# Autodesk Inventor assembly: Vergaser_ra8846s
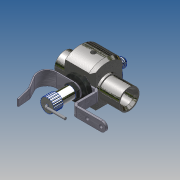
[picture p0: Inventor's stored thumbnail of the model, 180x180]
Saved by Autodesk Inventor 2021 (Build 250183000, 183)
## iProperties
Created: 2021-01-14
Part Number: Vergaser_ra8846s
Document SubType Name: Assembly
Designer: Sander
Author: Sander
## Documents named in this file (11)
- C:\Users\ricar\OneDrive - Fachhochschule Aachen\Mechatronik I\CAD\INVENTOR\Proyectos\Daten\Vergaser_ra8846s.iam
- C:\Users\ricar\OneDrive - Fachhochschule Aachen\Mechatronik I\CAD\INVENTOR\Proyectos\Daten\Vergasergehäuse_ra8846s.ipt
- C:\Users\ricar\OneDrive - Fachhochschule Aachen\Mechatronik I\CAD\INVENTOR\Proyectos\Daten\Einspritzdüse_ra8846s.ipt
- C:\Users\ricar\OneDrive - Fachhochschule Aachen\Mechatronik I\CAD\INVENTOR\Proyectos\Daten\Schließbahn_ra8846s.ipt
- C:\Users\ricar\OneDrive - Fachhochschule Aachen\Mechatronik I\CAD\INVENTOR\Proyectos\Daten\Gashebel_ra8846s.ipt
- C:\Users\ricar\OneDrive - Fachhochschule Aachen\Mechatronik I\CAD\INVENTOR\Proyectos\Daten\Dichtrign_ra8846s.ipt
- C:\Users\ricar\OneDrive - Fachhochschule Aachen\Mechatronik I\CAD\INVENTOR\Proyectos\Daten\Deckel_ra8846s.ipt
- C:\Users\ricar\OneDrive - Fachhochschule Aachen\Mechatronik I\CAD\INVENTOR\Proyectos\Daten\Rastfeder_ra8846s.ipt
- C:\Users\ricar\OneDrive - Fachhochschule Aachen\Mechatronik I\CAD\INVENTOR\Proyectos\Daten\Mutter_ra8846s.ipt
- C:\Users\ricar\OneDrive - Fachhochschule Aachen\Mechatronik I\CAD\INVENTOR\Proyectos\Daten\Nadelhalter_ra8846s.ipt
- C:\Users\ricar\OneDrive - Fachhochschule Aachen\Mechatronik I\CAD\INVENTOR\Proyectos\Daten\Düsennadel_ra8846s.ipt
## Components (10 placed, 10 different names)
1. Vergasergehäuse_ra8846s:1 — Passend:1, Winkel:1, Winkel:2, Winkel:3
2. Einspritzdüse_ra8846s:1 — Passend:1, Einfügen:1
3. Schließbahn_ra8846s:1 — Einfügen:1, Passend:2
4. Gashebel_ra8846s:1 — Passend:2, Einfügen:2, Winkel:1
5. Dichtrign_ra8846s:1 — Einfügen:2, Einfügen:3
6. Deckel_ra8846s:1 — Einfügen:3, Einfügen:4
7. Rastfeder_ra8846s:1 — Einfügen:4, Winkel:2, Einfügen:5
8. Mutter_ra8846s:1 — Einfügen:5, Einfügen:6
9. Nadelhalter_ra8846s:1 — Einfügen:6, Passend:3
10. Düsennadel_ra8846s:1 — Passend:3, Winkel:3
## Relationships (12: Insert 6, Mate 3, Angle 3)
- Passend:1 [Mate]: Vergasergehäuse_ra8846s:1 ↔ Einspritzdüse_ra8846s:1
- Einfügen:1 [Insert]: Einspritzdüse_ra8846s:1 ↔ Schließbahn_ra8846s:1
- Passend:2 [Mate]: Schließbahn_ra8846s:1 ↔ Gashebel_ra8846s:1
- Einfügen:2 [Insert]: Gashebel_ra8846s:1 ↔ Dichtrign_ra8846s:1
- Einfügen:3 [Insert]: Dichtrign_ra8846s:1 ↔ Deckel_ra8846s:1
- Winkel:1 [Angle] (0 deg): Vergasergehäuse_ra8846s:1 ↔ Gashebel_ra8846s:1
- Einfügen:4 [Insert]: Deckel_ra8846s:1 ↔ Rastfeder_ra8846s:1
- Winkel:2 [Angle] (0 deg): Vergasergehäuse_ra8846s:1 ↔ Rastfeder_ra8846s:1
- Einfügen:5 [Insert]: Rastfeder_ra8846s:1 ↔ Mutter_ra8846s:1
- Einfügen:6 [Insert]: Mutter_ra8846s:1 ↔ Nadelhalter_ra8846s:1
- Passend:3 [Mate]: Nadelhalter_ra8846s:1 ↔ Düsennadel_ra8846s:1
- Winkel:3 [Angle] (-90 deg): Vergasergehäuse_ra8846s:1 ↔ Düsennadel_ra8846s:1
